# Autodesk Inventor assembly: M5 Screw with Tee Nut Reverse
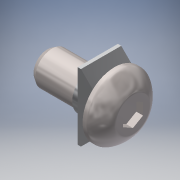
[picture p0: Inventor's stored thumbnail of the model, 180x180]
Saved by Autodesk Inventor 2017 (Build 210142000, 142)
## iProperties
Created: 2014-02-18
Part Number: M5 Screw with Tee Nut Reverse
Document SubType Name: Assembly
Designer: umr
Sending System: SolidWorks 2014
Last Author: Rory
Last Saved: 2016-05-20
Author: umr
## Documents named in this file (3)
- D:\SeniorProject\Models2\M5 Screw with Tee Nut Reverse.iam
- D:\SeniorProject\Models2\Tee Nut.ipt
- D:\SeniorProject\Models2\M5 Screw.ipt
## Components (2 placed, 2 different names)
1. Tee Nut:1 — Mate:1, Mate:2
2. M5 Screw:1 — Mate:1, Mate:2
## Relationships (2: Mate 2)
- Mate:1: Tee Nut:1 ↔ M5 Screw:1
- Mate:2: Tee Nut:1 ↔ M5 Screw:1
